# Autodesk Inventor assembly: MKPRO P1.2
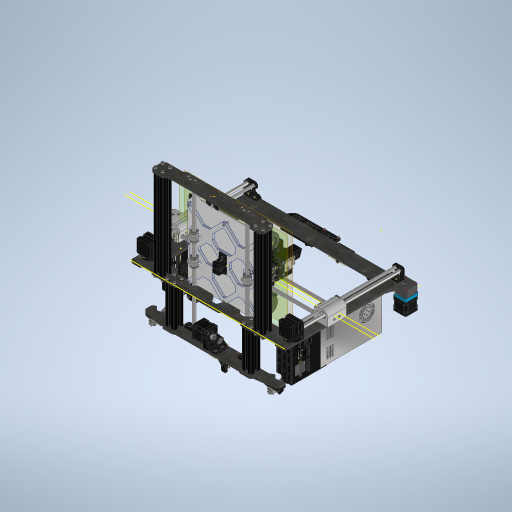
[picture p0: Inventor's stored thumbnail of the model, 512x512]
Saved by Autodesk Inventor 2023 (Build 270158000, 158)
## iProperties
Created: 2019-09-16
Part Number: MKPRO P1.2
Document SubType Name: Assembly
Designer: pepd9
Mass: 12945.6 g
Surface Area: 20679.4 cm^2
Volume: 3293.44 cm^3
Density: 3.93074 g/cm^3
Author: pepd9
## Documents named in this file (11)
- D:\000 - PEPCORP CLOUD\00- Legacy\Designs\MK3PRO P1\MKPRO P1.2.iam
- D:\000 - PEPCORP CLOUD\00- Legacy\Designs\MK3PRO P1\FRAME\Frame.iam
- D:\000 - PEPCORP CLOUD\00- Legacy\Designs\MK3PRO P1\Y-Axis\Y-AXIS ASSEMBLY P1.2.iam
- D:\000 - PEPCORP CLOUD\00- Legacy\Designs\MK3PRO P1\PSU\POWER.iam
- D:\000 - PEPCORP CLOUD\00- Legacy\Designs\MK3PRO P1\Z-Axis\Z-AXIS ASSEMBLY.iam
- D:\000 - PEPCORP CLOUD\00- Legacy\Designs\MK3PRO P1\X-Axis\X-AXIS ASSEMBLY.iam
- D:\000 - PEPCORP CLOUD\00- Legacy\Designs\MK3PRO P1\ELECTRONICS\Motherboard.iam
- D:\000 - PEPCORP CLOUD\00- Legacy\Designs\MK3PRO P1\E-Axis\E-AXIS ASSEMBLY P1.2.iam
- D:\000 - PEPCORP CLOUD\00- Legacy\Designs\MK3PRO P1\BED ASSEMBLY\Bed Assembly.iam
- D:\000 - PEPCORP CLOUD\00- Legacy\Designs\MK3PRO P1\E2\BowdenDriver.iam
- D:\000 - PEPCORP CLOUD\00- Legacy\Designs\MK3PRO P1\MKPRO P1.2_Substitute_1.ipt
## Components (9 placed, 9 different names)
1. Frame:1 [sub-assembly] — Flush:1, Flush:2, Flush:3, Mate:1, Mate:2, Mate:3, Mate:6, Mate:7, Mate:8, Mate:9, Mate:10, Mate:11, Mate:34, Mate:35, Mate:36, Mate:37, Mate:38, Mate:40, Mate:41, Mate:42, Mate:43, Mate:46, Mate:47
2. Y-AXIS ASSEMBLY P1.2:1 [sub-assembly] — Mate:1, Mate:2, Mate:3, Mate:44, Mate:45
3. POWER:1 [sub-assembly] — Mate:6, Mate:7, Mate:8
4. Z-AXIS ASSEMBLY:1 [sub-assembly] — Mate:9, Mate:10, Mate:11, Mate:48, Mate:49, Mate:50, Mate:51
5. Motherboard:1 [sub-assembly] — Mate:34, Mate:35, Mate:36, Mate:37, Mate:38, Mate:40, Mate:41, Mate:42, Mate:43
6. E-AXIS ASSEMBLY P1.2:1 [sub-assembly] — Mate:24, Mate:25, Flush:4, Flush:5, Flush:6, Flush:7, Flush:9
7. Bed Assembly:1 [sub-assembly] — Mate:44, Mate:45
8. X-AXIS ASSEMBLY:1 [sub-assembly] — Mate:24, Mate:25, Mate:48, Mate:49, Mate:50, Mate:51
9. BowdenDriver:1 [sub-assembly] — Mate:46, Mate:47
## Relationships (37: Mate 28, Flush 9)
- Flush:1: Frame:1
- Flush:2: Frame:1
- Flush:3: Frame:1
- Mate:1: Frame:1 ↔ Y-AXIS ASSEMBLY P1.2:1
- Mate:2: Frame:1 ↔ Y-AXIS ASSEMBLY P1.2:1
- Mate:3: Frame:1 ↔ Y-AXIS ASSEMBLY P1.2:1
- Mate:6: Frame:1 ↔ POWER:1
- Mate:7: Frame:1 ↔ POWER:1
- Mate:8: Frame:1 ↔ POWER:1
- Mate:9: Frame:1 ↔ Z-AXIS ASSEMBLY:1
- Mate:10: Frame:1 ↔ Z-AXIS ASSEMBLY:1
- Mate:11: Frame:1 ↔ Z-AXIS ASSEMBLY:1
- Mate:24: E-AXIS ASSEMBLY P1.2:1 ↔ X-AXIS ASSEMBLY:1
- Mate:25: E-AXIS ASSEMBLY P1.2:1 ↔ X-AXIS ASSEMBLY:1
- Mate:34: Frame:1 ↔ Motherboard:1
- Mate:35: Frame:1 ↔ Motherboard:1
- Mate:36: Frame:1 ↔ Motherboard:1
- Mate:37: Frame:1 ↔ Motherboard:1
- Mate:38: Frame:1 ↔ Motherboard:1
- Mate:40: Frame:1 ↔ Motherboard:1
- Mate:41: Frame:1 ↔ Motherboard:1
- Mate:42: Frame:1 ↔ Motherboard:1
- Mate:43: Frame:1 ↔ Motherboard:1
- Mate:44: Y-AXIS ASSEMBLY P1.2:1 ↔ Bed Assembly:1
- Mate:45: Y-AXIS ASSEMBLY P1.2:1 ↔ Bed Assembly:1
- Mate:46: Frame:1 ↔ BowdenDriver:1
- Mate:47: Frame:1 ↔ BowdenDriver:1
- Mate:48: Z-AXIS ASSEMBLY:1 ↔ X-AXIS ASSEMBLY:1
- Mate:49: Z-AXIS ASSEMBLY:1 ↔ X-AXIS ASSEMBLY:1
- Mate:50: Z-AXIS ASSEMBLY:1 ↔ X-AXIS ASSEMBLY:1
- Mate:51: Z-AXIS ASSEMBLY:1 ↔ X-AXIS ASSEMBLY:1
- Flush:4: E-AXIS ASSEMBLY P1.2:1
- Flush:5: E-AXIS ASSEMBLY P1.2:1
- Flush:6: E-AXIS ASSEMBLY P1.2:1
- Flush:7: E-AXIS ASSEMBLY P1.2:1
- Flush:8 (1.5 mm)
- Flush:9: E-AXIS ASSEMBLY P1.2:1
